# Autodesk Inventor assembly: something
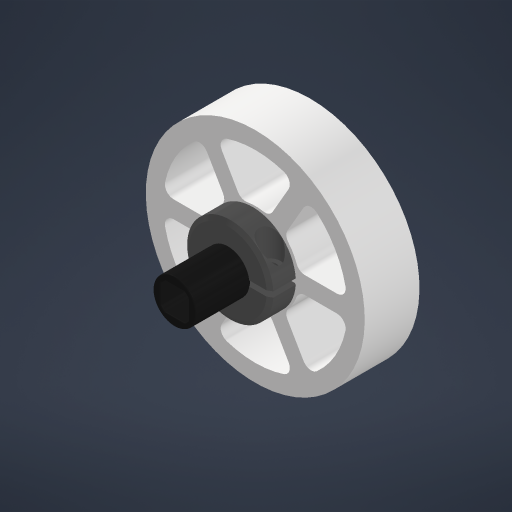
[picture p0: Inventor's stored thumbnail of the model, 512x512]
Saved by Autodesk Inventor 2023.4 (Build 274418000, 418)
## iProperties
Created: 2024-01-01
Part Number: something
Document SubType Name: Assembly
Designer: Meer
Author: Meer
## Documents named in this file (6)
- C:\Users\Meer\OneDrive\Documents\GitHub\2024-599Z\Cad\NEW Intake\something.iam
- C:\Users\Meer\OneDrive\Documents\GitHub\2024-599Z\Cad\Library\VEX-CAD-Inventor-1.4.0\Motion\Wheels\Flex Wheels\2.000 Flex Wheel\2.000 30A .500.ipt
- C:\Users\Meer\OneDrive\Documents\GitHub\2024-599Z\Cad\Library\VEX-CAD-Inventor-1.4.0\Motion\Wheels\Flex Wheels\2.000 Flex Wheel.ipt
- C:\Users\Meer\OneDrive\Documents\GitHub\2024-599Z\Cad\Library\VEX-CAD-Inventor-1.4.0\Motion\Shaft HS\HS Spacer\HSpacer .5000.ipt
- C:\Users\Meer\OneDrive\Documents\GitHub\2024-599Z\Cad\Library\VEX-CAD-Inventor-1.4.0\Motion\Shaft HS\HS Spacer.ipt
- C:\Users\Meer\OneDrive\Documents\GitHub\2024-599Z\Cad\Library\VEX-CAD-Inventor-1.4.0\Motion\Shaft HS\Low Profile HS Shaft Collar.ipt
## Components (5 placed, 3 different names)
1. 2.000 30A .500:1
2. HSpacer .5000:1 — Insert:1, Insert:2
3. Low Profile HS Shaft Collar:1 — Insert:1
4. Low Profile HS Shaft Collar:2 — Insert:2, Insert:3
5. HSpacer .5000:2 — Insert:3
## Relationships (3: Insert 3)
- Insert:1: HSpacer .5000:1 ↔ Low Profile HS Shaft Collar:1
- Insert:2: HSpacer .5000:1 ↔ Low Profile HS Shaft Collar:2
- Insert:3: Low Profile HS Shaft Collar:2 ↔ HSpacer .5000:2
